# Autodesk Inventor assembly: Thrust_Measure_Ball_Simulation
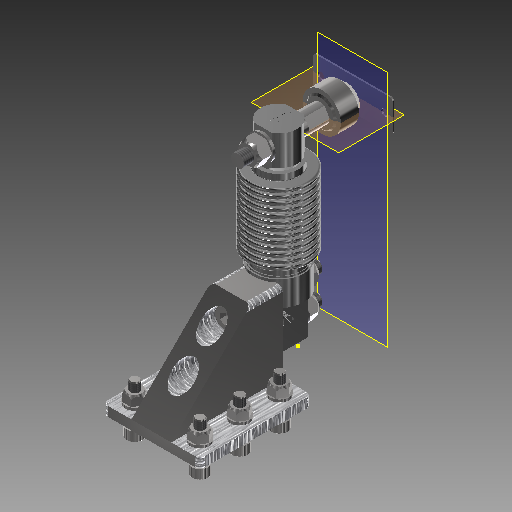
[picture p0: Inventor's stored thumbnail of the model, 512x512]
Saved by Autodesk Inventor 2019 (Build 230136000, 136)
## iProperties
Created: 2021-03-16
Part Number: Thrust_Measure_Ball_Simulation
Document SubType Name: Assembly
Designer: rtavi
Mass: 1064.54 g
Surface Area: 698.589 cm^2
Volume: 179.712 cm^3
Density: 5.92359 g/cm^3
Author: rtavi
## Documents named in this file (18)
- C:\Users\rtavi\Desktop\Uni\TFG\TestRig\Thrust_Measure.iam
- C:\Users\rtavi\Desktop\Uni\TFG\TestRig\CommercialParts\Load_Cell.ipt
- C:\Users\rtavi\Desktop\Uni\TFG\TestRig\DesignedParts\M6_M8_Adapter.ipt
- C:\Users\rtavi\Desktop\Uni\TFG\TestRig\CommercialParts\ball_unit_11mi-16-13.ipt
- C:\Users\rtavi\Desktop\Uni\TFG\TestRig\DesignedParts\LC_Support.ipt
- C:\Users\rtavi\Desktop\Uni\TFG\TestRig\CommercialParts\Screws\m6x25.ipt
- C:\Users\rtavi\Desktop\Uni\TFG\TestRig\CommercialParts\Screws\m6-washer.ipt
- C:\Users\rtavi\Desktop\Uni\TFG\TestRig\CommercialParts\Screws\m6-nut.ipt
- C:\Users\rtavi\Desktop\Uni\TFG\TestRig\DesignedParts\Hardened_Plate.ipt
- C:\Users\rtavi\Desktop\Uni\TFG\TestRig\CommercialParts\Screws\m8x50.ipt
- C:\Users\rtavi\Desktop\Uni\TFG\TestRig\CommercialParts\Screws\m8-nut.ipt
- C:\Users\rtavi\Desktop\Uni\TFG\TestRig\CommercialParts\Screws\m8-washer.ipt
- C:\Users\rtavi\Desktop\Uni\TFG\TestRig\SimulationFiles\dk0zoe5cw.fins
- C:\Users\rtavi\Desktop\Uni\TFG\TestRig\SimulationFiles\dk0zoe5cw.fsat
- C:\Users\rtavi\Desktop\Uni\TFG\TestRig\SimulationFiles\dk0zoe5cw.ftes
- C:\Users\rtavi\Desktop\Uni\TFG\TestRig\SimulationFiles\dk0zoe5cw.fwiz
- C:\Users\rtavi\Desktop\Uni\TFG\TestRig\SimulationFiles\dk0zoe5kw.fmsh
- C:\Users\rtavi\Desktop\Uni\TFG\TestRig\SimulationFiles\dk0zoe5kx.fres
## Components (31 placed, 11 different names)
1. Load_Cell:1 — Mate:1, Flush:3, Flush:4, Mate:16, Mate:17, Mate:20, Flush:9, Mate:28, Mate:29, Mate:30, Mate:35, Mate:40
2. M6_M8_Adapter:1 — Mate:16, Mate:17, Mate:18, Mate:19, Mate:31, Mate:32
3. ball_unit_11mi-16-13:1 — Mate:18, Mate:19, Tangent:1
4. LC_Support:1 — Flush:5, Flush:6, Flush:7, Mate:20, Mate:21, Mate:22, Mate:24, Mate:27, Mate:38, Mate:39
5. Hardened_Plate:1 — Flush:8, Flush:9, Tangent:1
6. m8x50:1 — Mate:28, Mate:34, Mate:36, Mate:38
7. m8x50:2 — Mate:29, Mate:39, Mate:41, Mate:42
8. m8-nut:1 — Mate:32, Mate:33
9. m8-washer:1 — Mate:30, Mate:31, Mate:33
10. m8-nut:2 — Mate:36, Mate:37
11. m8-washer:2 — Mate:34, Mate:35, Mate:37
12. m8-nut:3 — Mate:42, Mate:43
13. m8-washer:3 — Mate:40, Mate:41, Mate:43
14. m6x25:1 — Mate:22, Mate:23, Mate:25, Mate:27
15. m6-nut:1 — Mate:25, Mate:26
16. m6-washer:1 — Mate:23, Mate:24, Mate:26
17. m6x25:2
18. m6-nut:2
19. m6-washer:2
20. m6x25:3
21. m6-nut:3
22. m6-washer:3
23. m6x25:4
24. m6-nut:4
25. m6-washer:4
26. m6x25:5
27. m6-nut:5
28. m6-washer:5
29. m6x25:6
30. m6-nut:6
31. m6-washer:6
## Component patterns: (6 elements, first: m6x25:1 + m6-nut:1 + m6-washer:1)
## Relationships (37: Mate 29, Flush 7, Tangent 1)
- Mate:1 (16 mm): Load_Cell:1
- Flush:3: Load_Cell:1
- Flush:4: Load_Cell:1
- Mate:16: Load_Cell:1 ↔ M6_M8_Adapter:1
- Mate:17: Load_Cell:1 ↔ M6_M8_Adapter:1
- Mate:18: M6_M8_Adapter:1 ↔ ball_unit_11mi-16-13:1
- Mate:19: M6_M8_Adapter:1 ↔ ball_unit_11mi-16-13:1
- Flush:5: LC_Support:1
- Flush:6: LC_Support:1
- Flush:7: LC_Support:1
- Mate:20: Load_Cell:1 ↔ LC_Support:1
- Mate:21: LC_Support:1
- Mate:22: LC_Support:1 ↔ m6x25:1
- Mate:23: m6x25:1 ↔ m6-washer:1
- Mate:24: LC_Support:1 ↔ m6-washer:1
- Mate:25: m6x25:1 ↔ m6-nut:1
- Mate:26: m6-nut:1 ↔ m6-washer:1
- Mate:27 (6 mm): LC_Support:1 ↔ m6x25:1
- Flush:8: Hardened_Plate:1
- Flush:9: Load_Cell:1 ↔ Hardened_Plate:1
- Tangent:1: ball_unit_11mi-16-13:1 ↔ Hardened_Plate:1
- Mate:28: Load_Cell:1 ↔ m8x50:1
- Mate:29: Load_Cell:1 ↔ m8x50:2
- Mate:30: Load_Cell:1 ↔ m8-washer:1
- Mate:31: M6_M8_Adapter:1 ↔ m8-washer:1
- Mate:32: M6_M8_Adapter:1 ↔ m8-nut:1
- Mate:33: m8-nut:1 ↔ m8-washer:1
- Mate:34: m8x50:1 ↔ m8-washer:2
- Mate:35: Load_Cell:1 ↔ m8-washer:2
- Mate:36: m8x50:1 ↔ m8-nut:2
- Mate:37: m8-nut:2 ↔ m8-washer:2
- Mate:38: LC_Support:1 ↔ m8x50:1
- Mate:39: LC_Support:1 ↔ m8x50:2
- Mate:40: Load_Cell:1 ↔ m8-washer:3
- Mate:41: m8x50:2 ↔ m8-washer:3
- Mate:42: m8x50:2 ↔ m8-nut:3
- Mate:43: m8-nut:3 ↔ m8-washer:3
## Named parameters: sa_0 = 50000
note: some values were not read from the file. Shown as the stored number, unit unknown: "sa_0".
